# Autodesk Inventor assembly: Button
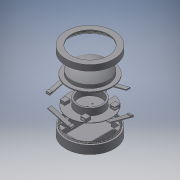
[picture p0: Inventor's stored thumbnail of the model, 180x180]
Saved by Autodesk Inventor 2016 SP2 (Build 200236200, 236)
## iProperties
Created: 2018-09-27
Part Number: Button
Material: Generisch
Document SubType Name: Assembly
Designer: Nils
Author: Nils
## Documents named in this file (7)
- C:\Users\Nils\Documents\Inventor\Bastelleien\Counter\Button\Button.iam
- C:\Users\Nils\Documents\Inventor\Bastelleien\Counter\Button\Bauteil1.ipt
- C:\Users\Nils\Documents\Inventor\Bastelleien\Counter\Button\Bauteil2.ipt
- C:\Users\Nils\Documents\Inventor\Bastelleien\Counter\Button\Spring.ipt
- C:\Users\Nils\Documents\Inventor\Bastelleien\Counter\Button\Spring2.ipt
- C:\Users\Nils\Documents\Inventor\Bastelleien\Counter\Button\Bauteil5.ipt
- C:\Users\Nils\Documents\Inventor\Bastelleien\Counter\Button\Bauteil6.ipt
## Components (9 placed, 6 different names)
1. Bauteil1:1 — Passend:2, Passend:3, Passend:4, Winkel:1, Passend:5, Passend:6, Passend:7, Passend:8, Passend:9, Passend:10, Passend:11, Passend:12, Passend:13, Passend:14, Passend:15, Passend:16, Passend:17, Passend:20, Passend:23
2. Bauteil2:1 — Passend:1, Passend:4, Passend:19, Passend:20, Passend:24
3. Spring:1 — Passend:5, Passend:6, Passend:13
4. Spring2:1 — Passend:21, Passend:22, Passend:23, Passend:24
5. Bauteil5:1 — Passend:1, Passend:3, Passend:18, Passend:19
6. Bauteil6:1 — Passend:2, Winkel:1, Passend:17, Passend:18, Passend:21, Passend:22
7. Spring:2 — Passend:9, Passend:10, Passend:15
8. Spring:3 — Passend:11, Passend:12, Passend:14
9. Spring:4 — Passend:7, Passend:8, Passend:16
## Relationships (25: Mate 24, Angle 1)
- Passend:1 [Mate]: Bauteil2:1 ↔ Bauteil5:1
- Passend:2 [Mate]: Bauteil1:1 ↔ Bauteil6:1
- Passend:3 [Mate]: Bauteil1:1 ↔ Bauteil5:1
- Passend:4 [Mate]: Bauteil1:1 ↔ Bauteil2:1
- Winkel:1 [Angle] (180 deg): Bauteil1:1 ↔ Bauteil6:1
- Passend:5 [Mate]: Bauteil1:1 ↔ Spring:1
- Passend:6 [Mate]: Bauteil1:1 ↔ Spring:1
- Passend:7 [Mate]: Bauteil1:1 ↔ Spring:4
- Passend:8 [Mate]: Bauteil1:1 ↔ Spring:4
- Passend:9 [Mate]: Bauteil1:1 ↔ Spring:2
- Passend:10 [Mate]: Bauteil1:1 ↔ Spring:2
- Passend:11 [Mate]: Bauteil1:1 ↔ Spring:3
- Passend:12 [Mate]: Bauteil1:1 ↔ Spring:3
- Passend:13 [Mate] (31.963 mm): Bauteil1:1 ↔ Spring:1
- Passend:14 [Mate] (36.579 mm): Bauteil1:1 ↔ Spring:3
- Passend:15 [Mate] (42.351 mm): Bauteil1:1 ↔ Spring:2
- Passend:16 [Mate] (45.387 mm): Bauteil1:1 ↔ Spring:4
- Passend:17 [Mate] (52.974 mm): Bauteil1:1 ↔ Bauteil6:1
- Passend:18 [Mate] (129.115 mm): Bauteil5:1 ↔ Bauteil6:1
- Passend:19 [Mate] (54.456 mm): Bauteil2:1 ↔ Bauteil5:1
- Passend:20 [Mate] (28.014 mm): Bauteil1:1 ↔ Bauteil2:1
- Passend:21 [Mate] (34 mm): Spring2:1 ↔ Bauteil6:1
- Passend:22 [Mate] (5 mm): Spring2:1 ↔ Bauteil6:1
- Passend:23 [Mate]: Bauteil1:1 ↔ Spring2:1
- Passend:24 [Mate] (51.5 mm): Bauteil2:1 ↔ Spring2:1
